# Autodesk Inventor assembly: WheelAssembly3.0
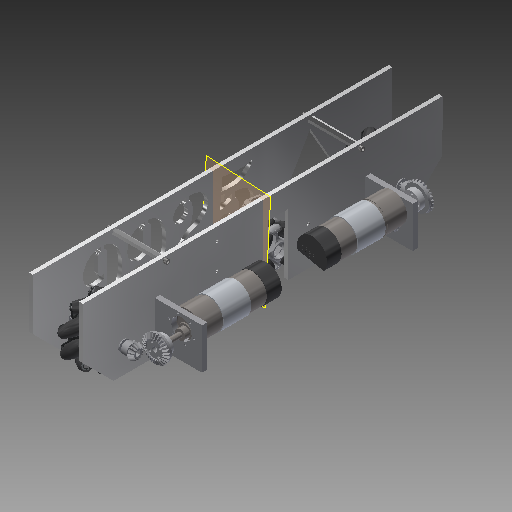
[picture p0: Inventor's stored thumbnail of the model, 512x512]
Saved by Autodesk Inventor 2019 (Build 230136000, 136)
## iProperties
Created: 2017-07-22
Part Number: WheelAssembly3.0
Document SubType Name: Assembly
Designer: User
Mass: 2301.48 g
Surface Area: 4071.67 cm^2
Volume: 902.346 cm^3
Density: 2.55055 g/cm^3
Author: User
## Documents named in this file (23)
- C:\Robotics\CAD\2020-21-CAD\Drivetrain\drive train left.iam
- C:\Robotics\CAD\2016-17_CAD\Custom COTS\4inax.ipt
- C:\Robotics\CAD\2018-19_CAD\Offseason\InvertedDrivePlateOutside.ipt
- C:\Robotics\CAD\2018-19_CAD\Offseason\InvertedDrivePlateInside.ipt
- C:\Robotics\CAD\COTSParts\Actobotics\535 parts\535198Bearing.25ID.5OD.ipt
- C:\Robotics\CAD\COTSParts\Actobotics\Collar.ipt
- C:\Robotics\CAD\COTSParts\Fasteners\6-32 SHCS x500.ipt
- C:\Robotics\CAD\COTSParts\Fasteners\Hex Standoff 6-32 x2250.ipt
- C:\Robotics\CAD\COTSParts\Motors\am-3102NeveRest20 (1)_MIR.ipt
- C:\Robotics\CAD\COTSParts\Rev\REV-41-1657MecanumWheelRight.iam
- C:\Robotics\CAD\2020-21-CAD\Drivetrain\motor mount.ipt
- C:\Robotics\CAD\COTSParts\Tetrix\Tetrix hub - motor.ipt
- C:\Robotics\CAD\2016-17_CAD\Custom COTS\4inax_MIR1.ipt
- C:\Robotics\CAD\COTSParts\Actobotics\535 parts\535198Bearing.25ID.5OD_MIR1.ipt
- C:\Robotics\CAD\COTSParts\Actobotics\Collar_MIR1.ipt
- C:\Robotics\CAD\COTSParts\Rev\REV-41-1657MecanumWheelRight_MIR.iam
- C:\Robotics\CAD\2020-21-CAD\Drivetrain\motor mount_MIR.ipt
- C:\Robotics\CAD\COTSParts\Motors\am-3102NeveRest20 (1)_MIR_MIR.ipt
- C:\Robotics\CAD\COTSParts\andymark\am-3902 am-3903 2in Omni 14mm Hex.ipt
- C:\Robotics\CAD\COTSParts\Rev\REV-11-1271.STEP encoders.ipt
- C:\Robotics\CAD\COTSParts\Actobotics\637 parts\637222 beval gear\615456 13tooth beval gear.ipt
- C:\Robotics\CAD\COTSParts\Actobotics\637 parts\637222 beval gear\615460 26 tooth beval gear.ipt
- C:\Robotics\CAD\COTSParts\Tetrix\Tetrix Hub - axle.ipt
## Components (39 placed, 22 different names)
1. 4inax:4 — Insert:147, Mate:63, Mate:69, Mate:101, Mate:102
2. InvertedDrivePlateOutside:1 — Flush:15, Mate:103, Flush:16, Mate:104, Mate:105, Mate:106, Mate:107, Angle:3, Mate:108, Mate:109
3. InvertedDrivePlateInside:1 — Insert:90, Insert:132, Insert:133, Insert:134, Insert:135, Insert:140, Insert:141, Insert:142, Insert:143, Flush:10, Flush:11, Angle:1, Mate:73, Mate:82, Mate:83, Flush:13, Mate:85, Mate:97, Flush:15, Flush:16
4. 535198Bearing.25ID.5OD:1 — Insert:86
5. Collar:1 — Insert:86, Insert:147
6. 535198Bearing.25ID.5OD:5 — Insert:90
7. Hex Standoff 6-32 x2250:1 — Insert:134, Mate:103
8. Hex Standoff 6-32 x2250:2 — Insert:132
9. Hex Standoff 6-32 x2250:3 — Insert:135
10. Hex Standoff 6-32 x2250:4 — Insert:133
11. 6-32 SHCS x500:22
12. 6-32 SHCS x500:23 — Mate:108, Mate:109
13. 6-32 SHCS x500:24
14. 6-32 SHCS x500:25
15. 6-32 SHCS x500:26 — Insert:140
16. 6-32 SHCS x500:27 — Insert:141
17. 6-32 SHCS x500:28 — Insert:142
18. 6-32 SHCS x500:29 — Insert:143
19. REV-41-1657MecanumWheelRight:1 [sub-assembly] — Mate:63, Mate:70, Mate:71, Mate:72, Flush:14
20. motor mount:1 — Flush:10, Mate:66, Mate:67, Flush:11, Flush:12, Mate:97, Mate:113
21. am-3102NeveRest20 (1)_MIR:2 — Mate:66, Mate:67, Angle:1, Angle:2, Mate:100, Mate:112
22. Tetrix hub - motor:1 — Mate:69, Mate:70, Mate:71, Mate:72, Mate:73
23. 4inax_MIR1:1 — Insert:150, Mate:76, Mate:92
24. 535198Bearing.25ID.5OD_MIR1:1 — Insert:151, Mate:105
25. Collar_MIR1:1 — Insert:150, Insert:151, Mate:104
26. 535198Bearing.25ID.5OD_MIR1:2 — Mate:82, Mate:83
27. REV-41-1657MecanumWheelRight_MIR:1 [sub-assembly] — Mate:76, Flush:14
28. motor mount_MIR:1 — Mate:78, Mate:79, Flush:12, Flush:13, Mate:85, Mate:95
29. am-3102NeveRest20 (1)_MIR_MIR:1 — Mate:78, Mate:79, Angle:2, Mate:96
30. am-3902 am-3903 2in Omni 14mm Hex:1 — Mate:89, Mate:90
31. REV-11-1271.STEP encoders:1 — Mate:89, Mate:90, Mate:106, Mate:107, Angle:3
32. 615456 13tooth beval gear:1 — Mate:92
33. 615460 26 tooth beval gear:1 — Mate:93, Mate:94, Mate:96
34. Tetrix Hub - axle:1 — Mate:93, Mate:94, Mate:95
35. 615456 13tooth beval gear:2 — Mate:101, Mate:102
36. 615460 26 tooth beval gear:2
37. Tetrix Hub - axle:2 — Mate:100
38. 615460 26 tooth beval gear:3 — Mate:113
39. Tetrix Hub - axle:3 — Mate:112
## Relationships (61: Mate 38, Insert 13, Flush 7, Angle 3)
- Insert:86: 535198Bearing.25ID.5OD:1 ↔ Collar:1
- Insert:90: InvertedDrivePlateInside:1 ↔ 535198Bearing.25ID.5OD:5
- Insert:132: InvertedDrivePlateInside:1 ↔ Hex Standoff 6-32 x2250:2
- Insert:133: InvertedDrivePlateInside:1 ↔ Hex Standoff 6-32 x2250:4
- Insert:134: InvertedDrivePlateInside:1 ↔ Hex Standoff 6-32 x2250:1
- Insert:135: InvertedDrivePlateInside:1 ↔ Hex Standoff 6-32 x2250:3
- Insert:140: InvertedDrivePlateInside:1 ↔ 6-32 SHCS x500:26
- Insert:141: InvertedDrivePlateInside:1 ↔ 6-32 SHCS x500:27
- Insert:142: InvertedDrivePlateInside:1 ↔ 6-32 SHCS x500:28
- Insert:143: InvertedDrivePlateInside:1 ↔ 6-32 SHCS x500:29
- Insert:147: 4inax:4 ↔ Collar:1
- Mate:63: 4inax:4 ↔ REV-41-1657MecanumWheelRight:1
- Flush:10 (88.9 mm): InvertedDrivePlateInside:1 ↔ motor mount:1
- Mate:66: motor mount:1 ↔ am-3102NeveRest20 (1)_MIR:2
- Mate:67: motor mount:1 ↔ am-3102NeveRest20 (1)_MIR:2
- Flush:11 (-12.7 mm): InvertedDrivePlateInside:1 ↔ motor mount:1
- Angle:1 (11.35 deg): InvertedDrivePlateInside:1 ↔ am-3102NeveRest20 (1)_MIR:2
- Mate:69: 4inax:4 ↔ Tetrix hub - motor:1
- Mate:70: REV-41-1657MecanumWheelRight:1 ↔ Tetrix hub - motor:1
- Mate:71: REV-41-1657MecanumWheelRight:1 ↔ Tetrix hub - motor:1
- Mate:72: REV-41-1657MecanumWheelRight:1 ↔ Tetrix hub - motor:1
- Mate:73 (19.05 mm): InvertedDrivePlateInside:1 ↔ Tetrix hub - motor:1
- Insert:150: 4inax_MIR1:1 ↔ Collar_MIR1:1
- Insert:151: 535198Bearing.25ID.5OD_MIR1:1 ↔ Collar_MIR1:1
- Mate:76: 4inax_MIR1:1 ↔ REV-41-1657MecanumWheelRight_MIR:1
- Mate:78: motor mount_MIR:1 ↔ am-3102NeveRest20 (1)_MIR_MIR:1
- Mate:79: motor mount_MIR:1 ↔ am-3102NeveRest20 (1)_MIR_MIR:1
- Mate:82: InvertedDrivePlateInside:1 ↔ 535198Bearing.25ID.5OD_MIR1:2
- Mate:83: InvertedDrivePlateInside:1 ↔ 535198Bearing.25ID.5OD_MIR1:2
- Flush:12: motor mount:1 ↔ motor mount_MIR:1
- Flush:13 (-88.9 mm): InvertedDrivePlateInside:1 ↔ motor mount_MIR:1
- Mate:85: InvertedDrivePlateInside:1 ↔ motor mount_MIR:1
- Angle:2 (0 deg): am-3102NeveRest20 (1)_MIR:2 ↔ am-3102NeveRest20 (1)_MIR_MIR:1
- Flush:14: REV-41-1657MecanumWheelRight:1 ↔ REV-41-1657MecanumWheelRight_MIR:1
- Mate:89: am-3902 am-3903 2in Omni 14mm Hex:1 ↔ REV-11-1271.STEP encoders:1
- Mate:90: am-3902 am-3903 2in Omni 14mm Hex:1 ↔ REV-11-1271.STEP encoders:1
- Mate:92: 4inax_MIR1:1 ↔ 615456 13tooth beval gear:1
- Mate:93: 615460 26 tooth beval gear:1 ↔ Tetrix Hub - axle:1
- Mate:94: 615460 26 tooth beval gear:1 ↔ Tetrix Hub - axle:1
- Mate:95 (19.05 mm): motor mount_MIR:1 ↔ Tetrix Hub - axle:1
- Mate:96: am-3102NeveRest20 (1)_MIR_MIR:1 ↔ 615460 26 tooth beval gear:1
- Mate:97: InvertedDrivePlateInside:1 ↔ motor mount:1
- [Mate]: 615460 26 tooth beval gear:2 ↔ Tetrix Hub - axle:2
- [Mate]: 615460 26 tooth beval gear:2 ↔ Tetrix Hub - axle:2
- Mate:100: am-3102NeveRest20 (1)_MIR:2 ↔ Tetrix Hub - axle:2
- Mate:101: 4inax:4 ↔ 615456 13tooth beval gear:2
- Mate:102: 4inax:4 ↔ 615456 13tooth beval gear:2
- Flush:15: InvertedDrivePlateOutside:1 ↔ InvertedDrivePlateInside:1
- Mate:103: InvertedDrivePlateOutside:1 ↔ Hex Standoff 6-32 x2250:1
- Flush:16: InvertedDrivePlateOutside:1 ↔ InvertedDrivePlateInside:1
- Mate:104: InvertedDrivePlateOutside:1 ↔ Collar_MIR1:1
- Mate:105: InvertedDrivePlateOutside:1 ↔ 535198Bearing.25ID.5OD_MIR1:1
- Mate:106: InvertedDrivePlateOutside:1 ↔ REV-11-1271.STEP encoders:1
- Mate:107: InvertedDrivePlateOutside:1 ↔ REV-11-1271.STEP encoders:1
- Angle:3 (-30 deg): InvertedDrivePlateOutside:1 ↔ REV-11-1271.STEP encoders:1
- Mate:108: InvertedDrivePlateOutside:1 ↔ 6-32 SHCS x500:23
- Mate:109: InvertedDrivePlateOutside:1 ↔ 6-32 SHCS x500:23
- [Mate]: 615460 26 tooth beval gear:3 ↔ Tetrix Hub - axle:3
- [Mate]: 615460 26 tooth beval gear:3 ↔ Tetrix Hub - axle:3
- Mate:112: am-3102NeveRest20 (1)_MIR:2 ↔ Tetrix Hub - axle:3
- Mate:113 (25.4 mm): motor mount:1 ↔ 615460 26 tooth beval gear:3
## Named parameters: d366_d360 = 0 mm, d367_d361 = 0 mm, d382_d360 = 0 mm, d383_d361 = 0 mm
